# Autodesk Inventor assembly: Ensamblaje_soportme molde_barras
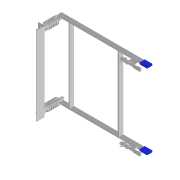
[picture p0: Inventor's stored thumbnail of the model, 180x180]
Saved by Autodesk Inventor 2021 (Build 250183000, 183)
## iProperties
Created: 2021-04-17
Part Number: Ensamblaje_soportme molde_barras
Document SubType Name: Assembly
Designer: Admin
Author: Admin
## Documents named in this file (8)
- C:\Users\carlo\Desktop\01 CAD\Ensamblaje_soportme molde_barras.iam
- C:\Users\carlo\Desktop\01 CAD\Soporte_molde.ipt
- C:\Users\carlo\Desktop\01 CAD\Mangas_soporte_molde.ipt
- C:\Users\carlo\Desktop\01 CAD\Toggle_clamp.iam
- C:\Users\carlo\Desktop\01 CAD\Barra_circular_soporte.ipt
- C:\Users\carlo\Desktop\01 CAD\Resorte_soporte_ material.ipt
- C:\Users\carlo\Desktop\01 CAD\perfil_fijacion.ipt
- C:\Users\carlo\Desktop\01 CAD\Pin_soporte.ipt
## Components (12 placed, 7 different names)
1. Soporte_molde:1 — Coincidencia:1, Coincidencia:2, Coincidencia:3, Coincidencia:4, Coincidencia:5, Coincidencia:6, Coincidencia:7, Coincidencia:8, De rotación:1, De rotación:2, Coincidencia:14
2. Mangas_soporte_molde:1 — Coincidencia:1, Coincidencia:2, Coincidencia:3
3. Mangas_soporte_molde:2 — Coincidencia:4, Coincidencia:5, Coincidencia:6
4. Toggle_clamp:1 [sub-assembly] — Coincidencia:7
5. Toggle_clamp:2 [sub-assembly] — Coincidencia:8
6. Barra_circular_soporte:1 — De rotación:1, Coincidencia:16, Coincidencia:18
7. Barra_circular_soporte:2 — De rotación:2, Coincidencia:12, Coincidencia:13, Coincidencia:15, Coincidencia:17
8. Resorte_soporte_ material:1 — Coincidencia:12
9. Resorte_soporte_ material:2 — Coincidencia:16
10. perfil_fijacion:1 — Coincidencia:13, Coincidencia:14, Coincidencia:15
11. Pin_soporte:1 — Coincidencia:17
12. Pin_soporte:2 — Coincidencia:18
## Relationships (17: Mate 15, RevoluteJoint 2)
- Coincidencia:1 [Mate]: Soporte_molde:1 ↔ Mangas_soporte_molde:1
- Coincidencia:2 [Mate]: Soporte_molde:1 ↔ Mangas_soporte_molde:1
- Coincidencia:3 [Mate]: Soporte_molde:1 ↔ Mangas_soporte_molde:1
- Coincidencia:4 [Mate]: Soporte_molde:1 ↔ Mangas_soporte_molde:2
- Coincidencia:5 [Mate]: Soporte_molde:1 ↔ Mangas_soporte_molde:2
- Coincidencia:6 [Mate]: Soporte_molde:1 ↔ Mangas_soporte_molde:2
- Coincidencia:7 [Mate]: Soporte_molde:1 ↔ Toggle_clamp:1
- Coincidencia:8 [Mate]: Soporte_molde:1 ↔ Toggle_clamp:2
- De rotación:1 [RevoluteJoint]: Soporte_molde:1 ↔ Barra_circular_soporte:1
- De rotación:2 [RevoluteJoint]: Soporte_molde:1 ↔ Barra_circular_soporte:2
- Coincidencia:12 [Mate]: Barra_circular_soporte:2 ↔ Resorte_soporte_ material:1
- Coincidencia:13 [Mate]: Barra_circular_soporte:2 ↔ perfil_fijacion:1
- Coincidencia:14 [Mate] (100 mm): Soporte_molde:1 ↔ perfil_fijacion:1
- Coincidencia:15 [Mate]: Barra_circular_soporte:2 ↔ perfil_fijacion:1
- Coincidencia:16 [Mate]: Barra_circular_soporte:1 ↔ Resorte_soporte_ material:2
- Coincidencia:17 [Mate]: Barra_circular_soporte:2 ↔ Pin_soporte:1
- Coincidencia:18 [Mate]: Barra_circular_soporte:1 ↔ Pin_soporte:2
